# Autodesk Inventor assembly: Top Bar
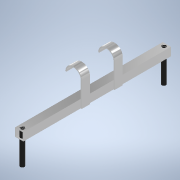
[picture p0: Inventor's stored thumbnail of the model, 180x180]
Saved by Autodesk Inventor 2020 (Build 240168000, 168)
## iProperties
Created: 2020-01-30
Part Number: Top Bar
Document SubType Name: Assembly
Designer: autum
Author: autum
## Documents named in this file (4)
- C:\Users\autum\Google Drive\Iron Riders 4180 (Roosevelt Robotics)\2019-2020\Build_Design\Robot 2020 (1)\Climber\Top Bar.iam
- C:\Users\autum\Google Drive\Iron Riders 4180 (Roosevelt Robotics)\2019-2020\Build_Design\Robot 2020 (1)\Climber\Top Bar.ipt
- C:\Users\autum\Google Drive\Iron Riders 4180 (Roosevelt Robotics)\2019-2020\Build_Design\Robot 2020 (1)\Climber\Hook 2.0.ipt
- C:\Users\autum\Google Drive\Iron Riders 4180 (Roosevelt Robotics)\2019-2020\Build_Design\Robot 2020 (1)\Climber\Insert.ipt
## Components (5 placed, 3 different names)
1. Top Bar:1 — Mate:1, Mate:2, Flush:1, Flush:2, Flush:3, Flush:4, Flush:5, Mate:4, Mate:5, Mate:6, Mate:7
2. Hook 2.0:1 — Mate:1, Flush:2, Mate:3
3. Hook 2.0:2 — Mate:2, Flush:1, Mate:3, Flush:3
4. Insert:1 — Flush:4, Mate:4, Mate:5
5. Insert:2 — Flush:5, Mate:6, Mate:7
## Relationships (12: Mate 7, Flush 5)
- Mate:1: Top Bar:1 ↔ Hook 2.0:1
- Mate:2: Top Bar:1 ↔ Hook 2.0:2
- Flush:1: Top Bar:1 ↔ Hook 2.0:2
- Flush:2: Top Bar:1 ↔ Hook 2.0:1
- Mate:3 (76.2 mm): Hook 2.0:1 ↔ Hook 2.0:2
- Flush:3 (177.8 mm): Top Bar:1 ↔ Hook 2.0:2
- Flush:4: Top Bar:1 ↔ Insert:1
- Flush:5: Top Bar:1 ↔ Insert:2
- Mate:4 (-9.525 mm): Top Bar:1 ↔ Insert:1
- Mate:5 (-12.7 mm): Top Bar:1 ↔ Insert:1
- Mate:6 (-9.525 mm): Top Bar:1 ↔ Insert:2
- Mate:7 (-12.7 mm): Top Bar:1 ↔ Insert:2
